# Autodesk Inventor assembly: allbody
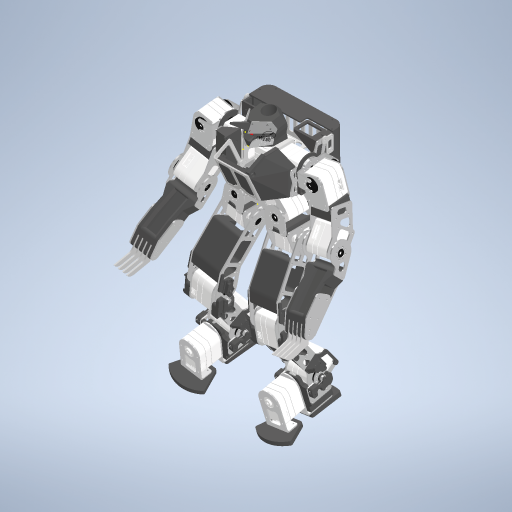
[picture p0: Inventor's stored thumbnail of the model, 512x512]
Saved by Autodesk Inventor 2024.1 (Build 281209000, 209)
## iProperties
Created: 2024-02-14
Part Number: allbody
Document SubType Name: Assembly
Designer: hibik
Author: hibik
## Documents named in this file (3)
- C:\Users\hibik\Desktop\ロボメカ\HR\2024.02.11 Rl\02.11 ProtType\allbody.iam
- C:\Users\hibik\Desktop\ロボメカ\HR\2024.02.11 Rl\02.11 ProtType\under_body.iam
- C:\Users\hibik\Desktop\ロボメカ\HR\2024.02.11 Rl\02.11 ProtType\upper_body.iam
## Components (2 placed, 2 different names)
1. under_body:1 [sub-assembly] — 挿入:1
2. upper_body:1 [sub-assembly] — 挿入:1
## Relationships (1: Insert 1)
- 挿入:1 [Insert] (0.3 mm): under_body:1 ↔ upper_body:1
